# Autodesk Inventor assembly: DSASSS
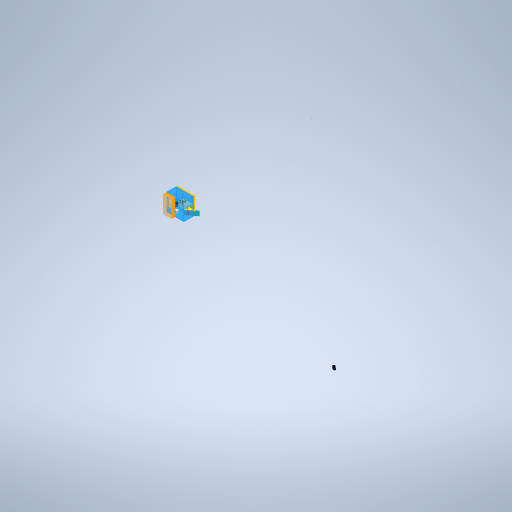
[picture p0: Inventor's stored thumbnail of the model, 512x512]
Saved by Autodesk Inventor 2024 (Build 280153000, 153)
## iProperties
Created: 2023-06-04
Part Number: DSASSS
Document SubType Name: Assembly
Designer: hithi
Author: hithi
## Documents named in this file (16)
- C:\Users\hithi\OneDrive\Desktop\DS\DSASSS.iam
- C:\Users\hithi\OneDrive\Desktop\DS\MAIN BODY.ipt
- C:\Users\hithi\OneDrive\Desktop\DS\ENTRY compartment.ipt
- C:\Users\hithi\Downloads\Ultra Sonic Sensor\Ultra Sonic Sensor.ipt
- C:\Users\hithi\Downloads\SPUR_06.ipt
- C:\Users\hithi\Downloads\RACK_06.ipt
- C:\Users\hithi\OneDrive\Desktop\DS\DSNDOOR 1.ipt
- C:\Users\hithi\OneDrive\Desktop\DS\bottom for door wheels.ipt
- C:\Users\hithi\Downloads\arduino_MEGA2650\arduino_MEGA2650.iam
- C:\Users\hithi\Downloads\Standard Large Breadboard with Two Side Rail\Standard Large Breadboard with Two Side Rail.iam
- C:\Users\hithi\Downloads\led-green-5mm-1.snapshot.1\BTG_901_BT_003_LED_5mm_Green\LED_5mm_Green.ipt
- C:\Users\hithi\Downloads\led-red-5mm-2.snapshot.1\BTG_901_BT_001_LED_5mm_Rot\LED_5mm_Rot.ipt
- C:\Users\hithi\Downloads\SG90_SG90\SG90_SG90.ipt
- C:\Users\hithi\OneDrive\Desktop\Part422.ipt
- C:\Users\hithi\OneDrive\Desktop\abcd.ipt
- C:\Users\hithi\OneDrive\Desktop\DS\CIRCUIT compartment.ipt
## Components (17 placed, 15 different names)
1. MAIN BODY:1 — Mate:1, Mate:2, Mate:3, Mate:4, Mate:6, Mate:7
2. ENTRY compartment:1 — Mate:1, Mate:2, Flush:1, Mate:5
3. Ultra Sonic Sensor:1 — Flush:1
4. SPUR_06:1
5. SPUR_06:1 — Mate:3, Mate:4
6. RACK_06:1 — Mate:5
7. DSNDOOR 1:1 — Mate:6, Mate:7
8. bottom for door wheels:1
9. arduino_MEGA2650:1 [sub-assembly]
10. Ultra Sonic Sensor:2
11. Standard Large Breadboard with Two Side Rail:1 [sub-assembly]
12. LED_5mm_Green:1
13. LED_5mm_Rot:1
14. SG90_SG90:1
15. Part422:1
16. abcd:1
17. CIRCUIT compartment:1
## Relationships (8: Mate 7, Flush 1)
- Mate:1: MAIN BODY:1 ↔ ENTRY compartment:1
- Mate:2: MAIN BODY:1 ↔ ENTRY compartment:1
- Flush:1: ENTRY compartment:1 ↔ Ultra Sonic Sensor:1
- Mate:3: MAIN BODY:1 ↔ SPUR_06:1
- Mate:4: MAIN BODY:1 ↔ SPUR_06:1
- Mate:5: ENTRY compartment:1 ↔ RACK_06:1
- Mate:6: MAIN BODY:1 ↔ DSNDOOR 1:1
- Mate:7: MAIN BODY:1 ↔ DSNDOOR 1:1
